# Autodesk Inventor assembly: WCP - Greyt Telescope (Stages 1-4)
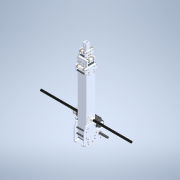
[picture p0: Inventor's stored thumbnail of the model, 180x180]
Saved by Autodesk Inventor 2022 (Build 260153000, 153)
## iProperties
Created: 2021-11-19
Part Number: WCP - Greyt Telescope (Stages 1-4)
Description: STEP AP214
Document SubType Name: Assembly
Designer: s143573
Sending System: SolidWorks 2020
Preprocessor: SwSTEP 2.0
Title: WCP - Greyt Telescope (Stages #1-4).step
Revision Number: ANY
## Documents named in this file (14)
- D:\STEP Files\Hardware\teleiscope arm\WCP - Greyt Telescope (Stages 1-4).iam
- D:\STEP Files\Hardware\teleiscope arm\WCP-0420-001 Rev1.ipt
- D:\STEP Files\Hardware\teleiscope arm\WCP-0420-002 Rev1.ipt
- D:\STEP Files\Hardware\teleiscope arm\WCP-0420-003 Rev1.ipt
- D:\STEP Files\Hardware\teleiscope arm\WCP-0420-004 Rev1.ipt
- D:\STEP Files\Hardware\teleiscope arm\WCP-0418 - TopBlock_2.iam
- D:\STEP Files\Hardware\teleiscope arm\WCP-0418 - BottomBlock_0.125_ Tubing.iam
- D:\STEP Files\Hardware\teleiscope arm\WCP-0419 - TopBlock_1.iam
- D:\STEP Files\Hardware\teleiscope arm\WCP-0419 - BottomBlock_0.125_ Tubing.iam
- D:\STEP Files\Hardware\teleiscope arm\WCP-0420 - TopBlock.iam
- D:\STEP Files\Hardware\teleiscope arm\WCP-0420 - BottomBlock_0.125_ Tubing.iam
- D:\STEP Files\Hardware\teleiscope arm\WCP-0416 - GreyT Telescope Gearbox (Stages #1-4)_2.5_ - Base Gearbox.iam
- D:\am-4124 500 Hex Hub.ipt
- D:\Arm shaft.ipt
## Components (15 placed, 13 different names)
1. WCP-0420-001 Rev1_12 — Mate:2, Mate:15, Mate:16, Mate:17, Angle:5, Angle:6, Tangent:5, Tangent:6, Mate:22, Mate:24, Mate:31, Mate:32, Mate:33, Mate:34
2. WCP-0420-002 Rev1_13 — Mate:3, Angle:3, Angle:4, Tangent:3, Tangent:4, Mate:14, Angle:5, Angle:6, Mate:18, Mate:19
3. WCP-0420-003 Rev1_14 — Mate:1, Angle:1, Angle:2, Mate:8, Mate:9, Tangent:1, Tangent:2, Mate:12, Mate:13, Angle:3, Angle:4
4. WCP-0420-004 Rev1_15 — Mate:7, Angle:1, Angle:2, Mate:10, Mate:11
5. WCP-0418 - TopBlock_16 [sub-assembly] — Mate:1, Mate:8, Mate:9
6. WCP-0418 - BottomBlock_0.125" Tubing_17 [sub-assembly] — Mate:7, Mate:10, Mate:11, Tangent:1, Tangent:2
7. WCP-0419 - TopBlock_18 [sub-assembly] — Mate:3, Mate:14
8. WCP-0419 - BottomBlock_0.125" Tubing_19 [sub-assembly] — Mate:12, Mate:13, Tangent:3, Tangent:4
9. WCP-0420 - TopBlock_20 [sub-assembly] — Mate:2
10. WCP-0420 - BottomBlock_0.125" Tubing_21 [sub-assembly] — Mate:18, Mate:19, Tangent:5, Tangent:6
11. WCP-0416 - GreyT Telescope Gearbox (Stages #1-4)_2.5" - Base Gearbox_45 [sub-assembly] — Mate:15, Mate:16, Mate:17
12. am-4124 500 Hex Hub:1 — Mate:22, Mate:25, Mate:26, Flush:1, Mate:31, Mate:33
13. am-4124 500 Hex Hub:2 — Mate:24, Mate:27, Mate:28, Mate:32, Mate:34, Flush:2
14. Arm shaft:1 — Mate:25, Mate:26, Flush:1
15. Arm shaft:2 — Mate:27, Mate:28, Flush:2
## Relationships (40: Mate 26, Angle 6, Tangent 6, Flush 2)
- Mate:1: WCP-0420-003 Rev1_14 ↔ WCP-0418 - TopBlock_16
- Mate:2: WCP-0420-001 Rev1_12 ↔ WCP-0420 - TopBlock_20
- Mate:3: WCP-0420-002 Rev1_13 ↔ WCP-0419 - TopBlock_18
- Mate:7: WCP-0420-004 Rev1_15 ↔ WCP-0418 - BottomBlock_0.125" Tubing_17
- Angle:1 (0 deg): WCP-0420-003 Rev1_14 ↔ WCP-0420-004 Rev1_15
- Angle:2 (0 deg): WCP-0420-003 Rev1_14 ↔ WCP-0420-004 Rev1_15
- Mate:8: WCP-0420-003 Rev1_14 ↔ WCP-0418 - TopBlock_16
- Mate:9: WCP-0420-003 Rev1_14 ↔ WCP-0418 - TopBlock_16
- Mate:10: WCP-0420-004 Rev1_15 ↔ WCP-0418 - BottomBlock_0.125" Tubing_17
- Mate:11: WCP-0420-004 Rev1_15 ↔ WCP-0418 - BottomBlock_0.125" Tubing_17
- Tangent:1: WCP-0420-003 Rev1_14 ↔ WCP-0418 - BottomBlock_0.125" Tubing_17
- Tangent:2: WCP-0420-003 Rev1_14 ↔ WCP-0418 - BottomBlock_0.125" Tubing_17
- Mate:12: WCP-0420-003 Rev1_14 ↔ WCP-0419 - BottomBlock_0.125" Tubing_19
- Mate:13: WCP-0420-003 Rev1_14 ↔ WCP-0419 - BottomBlock_0.125" Tubing_19
- Angle:3 (0 deg): WCP-0420-002 Rev1_13 ↔ WCP-0420-003 Rev1_14
- Angle:4 (0 deg): WCP-0420-002 Rev1_13 ↔ WCP-0420-003 Rev1_14
- Tangent:3: WCP-0420-002 Rev1_13 ↔ WCP-0419 - BottomBlock_0.125" Tubing_19
- Tangent:4: WCP-0420-002 Rev1_13 ↔ WCP-0419 - BottomBlock_0.125" Tubing_19
- Mate:14: WCP-0420-002 Rev1_13 ↔ WCP-0419 - TopBlock_18
- Mate:15: WCP-0420-001 Rev1_12 ↔ WCP-0416 - GreyT Telescope Gearbox (Stages #1-4)_2.5" - Base Gearbox_45
- Mate:16: WCP-0420-001 Rev1_12 ↔ WCP-0416 - GreyT Telescope Gearbox (Stages #1-4)_2.5" - Base Gearbox_45
- Mate:17: WCP-0420-001 Rev1_12 ↔ WCP-0416 - GreyT Telescope Gearbox (Stages #1-4)_2.5" - Base Gearbox_45
- Angle:5 (0 deg): WCP-0420-001 Rev1_12 ↔ WCP-0420-002 Rev1_13
- Angle:6 (0 deg): WCP-0420-001 Rev1_12 ↔ WCP-0420-002 Rev1_13
- Mate:18: WCP-0420-002 Rev1_13 ↔ WCP-0420 - BottomBlock_0.125" Tubing_21
- Mate:19: WCP-0420-002 Rev1_13 ↔ WCP-0420 - BottomBlock_0.125" Tubing_21
- Tangent:5: WCP-0420-001 Rev1_12 ↔ WCP-0420 - BottomBlock_0.125" Tubing_21
- Tangent:6: WCP-0420-001 Rev1_12 ↔ WCP-0420 - BottomBlock_0.125" Tubing_21
- Mate:22: WCP-0420-001 Rev1_12 ↔ am-4124 500 Hex Hub:1
- Mate:24: WCP-0420-001 Rev1_12 ↔ am-4124 500 Hex Hub:2
- Mate:25: am-4124 500 Hex Hub:1 ↔ Arm shaft:1
- Mate:26: am-4124 500 Hex Hub:1 ↔ Arm shaft:1
- Mate:27: am-4124 500 Hex Hub:2 ↔ Arm shaft:2
- Mate:28: am-4124 500 Hex Hub:2 ↔ Arm shaft:2
- Flush:1: am-4124 500 Hex Hub:1 ↔ Arm shaft:1
- Mate:31: WCP-0420-001 Rev1_12 ↔ am-4124 500 Hex Hub:1
- Mate:32: WCP-0420-001 Rev1_12 ↔ am-4124 500 Hex Hub:2
- Mate:33: WCP-0420-001 Rev1_12 ↔ am-4124 500 Hex Hub:1
- Mate:34: WCP-0420-001 Rev1_12 ↔ am-4124 500 Hex Hub:2
- Flush:2: am-4124 500 Hex Hub:2 ↔ Arm shaft:2
